# Autodesk Inventor assembly: Siding
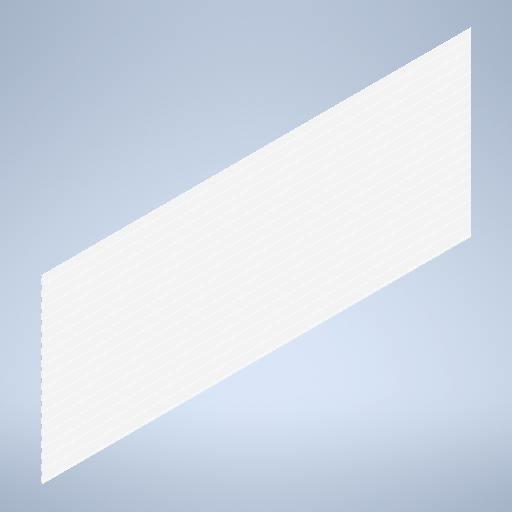
[picture p0: Inventor's stored thumbnail of the model, 512x512]
Saved by Autodesk Inventor 2025 (Build 290162010, 162A)
## iProperties
Created: 2024-09-16
Part Number: Siding
Document SubType Name: Assembly
Designer: Tom
Author: Tom
## Documents named in this file (3)
- C:\Users\Tom\Documents\Inventor\Mobility\Additional_Building\Siding_For_Back_Wall.iam
- C:\Users\Tom\Documents\Inventor\Mobility\Additional_Building\Starter_Strip_For_Back_Wall.ipt
- C:\Users\Tom\Documents\Inventor\Mobility\Additional_Building\Fiber_Cement_Board_For_Back_Wall.ipt
## Components (19 placed, 2 different names)
1. Starter_Strip_For_Back_Wall:1 — Mate:1, Mate:2, Flush:1, Flush:2, Mate:3
2. Fiber_Cement_Board_For_Back_Wall:1 — Mate:1, Mate:2, Flush:2, Mate:3
3. Fiber_Cement_Board_For_Back_Wall:2
4. Fiber_Cement_Board_For_Back_Wall:3
5. Fiber_Cement_Board_For_Back_Wall:4
6. Fiber_Cement_Board_For_Back_Wall:5
7. Fiber_Cement_Board_For_Back_Wall:6
8. Fiber_Cement_Board_For_Back_Wall:7
9. Fiber_Cement_Board_For_Back_Wall:8
10. Fiber_Cement_Board_For_Back_Wall:9
11. Fiber_Cement_Board_For_Back_Wall:10
12. Fiber_Cement_Board_For_Back_Wall:11
13. Fiber_Cement_Board_For_Back_Wall:12
14. Fiber_Cement_Board_For_Back_Wall:13
15. Fiber_Cement_Board_For_Back_Wall:14
16. Fiber_Cement_Board_For_Back_Wall:15
17. Fiber_Cement_Board_For_Back_Wall:16
18. Fiber_Cement_Board_For_Back_Wall:17
19. Fiber_Cement_Board_For_Back_Wall:18
## Component patterns: (18 elements, first: Fiber_Cement_Board_For_Back_Wall:1)
## Relationships (5: Mate 3, Flush 2)
- Mate:1: Starter_Strip_For_Back_Wall:1 ↔ Fiber_Cement_Board_For_Back_Wall:1
- Mate:2: Starter_Strip_For_Back_Wall:1 ↔ Fiber_Cement_Board_For_Back_Wall:1
- Flush:1: Starter_Strip_For_Back_Wall:1
- Flush:2: Starter_Strip_For_Back_Wall:1 ↔ Fiber_Cement_Board_For_Back_Wall:1
- Mate:3 (6.35 mm): Starter_Strip_For_Back_Wall:1 ↔ Fiber_Cement_Board_For_Back_Wall:1
